# Autodesk Inventor assembly: Fingertip assembly final
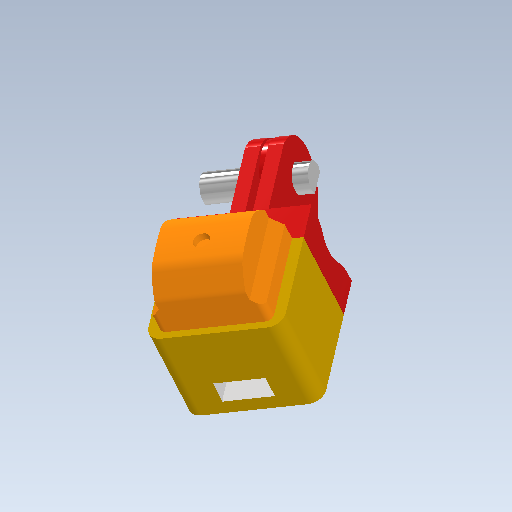
[picture p0: Inventor's stored thumbnail of the model, 512x512]
Saved by Autodesk Inventor 2020 (Build 240168000, 168)
## iProperties
Created: 2020-02-13
Part Number: Fingertip assembly final
Document SubType Name: Assembly
Designer: kaipa
Author: kaipa
## Documents named in this file (6)
- C:\Users\sami_\Documents\V1.6\Workgroups\NotInProject\PINKY\Fingertip assembly final.iam
- C:\Users\sami_\Documents\V1.6\Workgroups\NotInProject\PINKY\L3.ipt
- C:\Users\sami_\Documents\V1.6\Workgroups\NotInProject\PINKY\fingertip lid 5.ipt
- C:\Users\sami_\Documents\V1.6\Workgroups\NotInProject\1D Fingertip skeleton.ipt
- C:\Users\sami_\Documents\V1.6\Workgroups\NotInProject\SHAFT.ipt
- C:\Users\sami_\Documents\V1.6\Workgroups\NotInProject\Fingertiptest2-Solid 2mm base.ipt
## Components (6 placed, 5 different names)
1. L3:1 — Rigid:3, Rigid:5
2. fingertip lid 5:1
3. 1D Fingertip skeleton:1 — Rigid:3, Rigid:4
4. fingertip lid 5:2
5. SHAFT:1 — Rigid:5
6. Fingertiptest2-Solid 2mm base:2 — Rigid:4
## Relationships (5: WeldJoint 5)
- [WeldJoint]: fingertip lid 5:1 ↔ 1D Fingertip skeleton:1
- [WeldJoint]: 1D Fingertip skeleton:1 ↔ fingertip lid 5:2
- Rigid:3 [WeldJoint]: L3:1 ↔ 1D Fingertip skeleton:1
- Rigid:4 [WeldJoint] (-1 mm): 1D Fingertip skeleton:1 ↔ Fingertiptest2-Solid 2mm base:2
- Rigid:5 [WeldJoint] (2 mm): L3:1 ↔ SHAFT:1
